# Autodesk Inventor assembly: Assem1
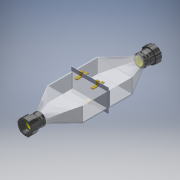
[picture p0: Inventor's stored thumbnail of the model, 180x180]
Saved by Autodesk Inventor 2017 (Build 210142000, 142)
## iProperties
Created: 2014-08-02
Part Number: Assem1
Document SubType Name: Assembly
Designer: XuZhiqing
Sending System: SolidWorks 2014
Last Author: 1
Last Saved: 2014-09-23
Author: XuZhiqing
## Documents named in this file (4)
- C:\Users\XuZhiqing\Desktop\Project01-APS490-CAD-CFD2\CAD-Whole Sys Final\filter and gauge\filter and gauge\filter and gauge.iam
- C:\Users\XuZhiqing\Desktop\Project01-APS490-CAD-CFD2\CAD-Whole Sys Final\filter and gauge\filter and gauge\Solid9.ipt
- C:\Users\XuZhiqing\Desktop\Project01-APS490-CAD-CFD2\CAD-Whole Sys Final\filter and gauge\filter\Assem1.iam
- C:\Users\XuZhiqing\Desktop\Project01-APS490-CAD-CFD2\CAD-Whole Sys Final\other\banjo female cam.ipt
## Components (4 placed, 3 different names)
1. Solid9:1
2. Assem1:1 [sub-assembly] — Angle:1, Mate:3, Mate:5
3. banjo female cam:1 — Angle:1, Mate:3, Mate:4
4. banjo female cam:2 — Mate:4, Mate:5
## Relationships (4: Mate 3, Angle 1)
- Angle:1 (180 deg): Assem1:1 ↔ banjo female cam:1
- Mate:3: Assem1:1 ↔ banjo female cam:1
- Mate:4: banjo female cam:1 ↔ banjo female cam:2
- Mate:5: Assem1:1 ↔ banjo female cam:2
